# Autodesk Inventor assembly: TC-R1 2×1 B
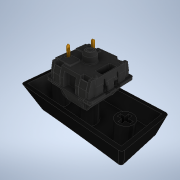
[picture p0: Inventor's stored thumbnail of the model, 180x180]
Saved by Autodesk Inventor 2020 (Build 240168000, 168)
## iProperties
Created: 2019-07-03
Part Number: TC-R1 2×1 B
Document SubType Name: Assembly
Designer: Thibault
Mass: 0.99122 g
Surface Area: 32.3296 cm^2
Volume: 0.99122 cm^3
Density: 1 g/cm^3
Author: Thibault
Sending System: Creo  TM  3.0
## Documents named in this file (10)
- C:\Users\Thibault Polge\Documents\Habilis\mech\mx\TC-R1 2×1 B.iam
- C:\Users\Thibault Polge\Documents\Habilis\mech\MX_DOWN.ipt
- C:\Users\Thibault Polge\Documents\Habilis\mech\MX_UP.ipt
- C:\Users\Thibault Polge\Documents\Habilis\mech\MX_PIN.ipt
- C:\Users\Thibault Polge\Documents\Habilis\mech\MX_SPRING.ipt
- C:\Users\Thibault Polge\Documents\Habilis\mech\MX_CLICK.ipt
- C:\Users\Thibault Polge\Documents\Habilis\mech\keycaps\1x2 R1 v6.ipt
- C:\Users\Thibault Polge\Documents\Habilis\mech\mx_stem\Brown.ipt
- C:\Users\Thibault Polge\Documents\Habilis\mech\mx_stem.ipt
- C:\Users\Thibault Polge\Documents\Habilis\mech\mx.iam
## Components (7 placed, 7 different names)
1. MX_DOWN — Placage:2
2. MX_UP — Placage:3, Angle:5
3. UP_MX — Placage:2, Placage:3, Placage:12, Placage:13
4. MX_PIN
5. MX_SPRING
6. MX_CLICK
7. 1x2 R1 v6:1 — Placage:12, Angle:5, Placage:13
## Relationships (5: Mate 4, Angle 1)
- Placage:2 [Mate]: MX_DOWN ↔ UP_MX
- Placage:3 [Mate]: MX_UP ↔ UP_MX
- Placage:12 [Mate]: UP_MX ↔ 1x2 R1 v6:1
- Angle:5 (0 deg): MX_UP ↔ 1x2 R1 v6:1
- Placage:13 [Mate]: UP_MX ↔ 1x2 R1 v6:1
